# Autodesk Inventor assembly: 63835A42
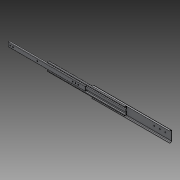
[picture p0: Inventor's stored thumbnail of the model, 180x180]
Saved by Autodesk Inventor 2014 SP1 (Build 180222100, 222)
## iProperties
Created: 2014-04-03
Part Number: 63835A42
Document SubType Name: Assembly
Designer: TDM
Mass: 92.0454 g
Surface Area: 1242.33 cm^2
Volume: 92.0454 cm^3
Density: 1 g/cm^3
VLDS_Profile: Default Assembly
VLDS_TimeStamp: 2014-04-11
VLDS_FailCnt: 0
VLDS_AcceptCnt: 0
Author: TDM
## Documents named in this file (4)
- C:\Users\TODD D MILLER\SkyDrive\TCM Design Group\GrabCAD\RABACONDA\PURCHASED\63835A42.iam
- C:\Users\TODD D MILLER\SkyDrive\TCM Design Group\GrabCAD\RABACONDA\PURCHASED\63835A420 BASE.ipt
- C:\Users\TODD D MILLER\SkyDrive\TCM Design Group\GrabCAD\RABACONDA\PURCHASED\63835A420 CENTER.ipt
- C:\Users\TODD D MILLER\SkyDrive\TCM Design Group\GrabCAD\RABACONDA\PURCHASED\63835A420 END.ipt
## Components (3 placed, 3 different names)
1. 63835A420 BASE:1 — Flush:1, Flush:2, Flush:3, Flush:4, Flush:5
2. 63835A420 CENTER:1 — Flush:1, Flush:2, Flush:5, Flush:6
3. 63835A420 END:1 — Flush:3, Flush:4, Flush:6
## Relationships (6: Flush 6)
- Flush:1: 63835A420 BASE:1 ↔ 63835A420 CENTER:1
- Flush:2: 63835A420 BASE:1 ↔ 63835A420 CENTER:1
- Flush:3: 63835A420 BASE:1 ↔ 63835A420 END:1
- Flush:4: 63835A420 BASE:1 ↔ 63835A420 END:1
- Flush:5 (204.1906 mm): 63835A420 BASE:1 ↔ 63835A420 CENTER:1
- Flush:6 (178.3334 mm): 63835A420 CENTER:1 ↔ 63835A420 END:1
